# Autodesk Inventor assembly: Assembly1
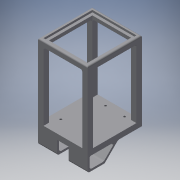
[picture p0: Inventor's stored thumbnail of the model, 180x180]
Saved by Autodesk Inventor 2016 (Build 200138000, 138)
## iProperties
Created: 2018-09-18
Part Number: Assembly1
Document SubType Name: Assembly
Designer: Kyle
Author: Kyle
## Documents named in this file (3)
- A:\Inventor current projects\PacBot\v.0.3.0\Assembly1.iam
- A:\Inventor current projects\PacBot\v.0.3.0\Base.ipt
- A:\Inventor current projects\PacBot\v.0.3.0\Hood_base.ipt
## Components (2 placed, 2 different names)
1. Base:1 — Mate:1, Flush:1, Flush:2
2. Hood_base:1 — Mate:1, Flush:1, Flush:2
## Relationships (3: Flush 2, Mate 1)
- Mate:1: Base:1 ↔ Hood_base:1
- Flush:1: Base:1 ↔ Hood_base:1
- Flush:2: Base:1 ↔ Hood_base:1
